# Autodesk Inventor assembly: 00_X02598_LEGOmini_CityGuy
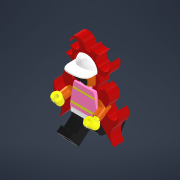
[picture p0: Inventor's stored thumbnail of the model, 180x180]
Saved by Autodesk Inventor 2022 (Build 260153000, 153)
## iProperties
Created: 2022-02-05
Part Number: 00_X02598_LEGOmini_CityGuy
Document SubType Name: Assembly
Designer: Jason
Author: Jason
## Documents named in this file (5)
- C:\Users\User\Desktop\教材_LEGOmini_2022_20220218\00_X02598_LEGOmini_CityGuy.iam
- C:\Users\User\Desktop\教材_LEGOmini_2022_20220218\X02598_LEGOmini_LowerBody.iam
- C:\Users\User\Desktop\教材_LEGOmini_2022_20220218\X02598_LEGOmini_UpperBody.iam
- C:\Users\User\Desktop\教材_LEGOmini_2022_20220218\X02598_LEGOmini_Head_Y.ipt
- C:\Users\User\Desktop\教材_LEGOmini_2022_20220218\X02598_LEGOmini_Hat_R.ipt
## Components (4 placed, 4 different names)
1. X02598_LEGOmini_LowerBody:1 [sub-assembly] — 貼合:1, 齊平:1, 齊平:2
2. X02598_LEGOmini_UpperBody:1 [sub-assembly] — 貼合:1, 齊平:1, 齊平:2, 插入:1, 齊平:3
3. X02598_LEGOmini_Head_Y:1 — 插入:1, 插入:2, 齊平:3
4. X02598_LEGOmini_Hat_R:1 — 插入:2
## Relationships (6: Flush 3, Insert 2, Mate 1)
- 貼合:1 [Mate]: X02598_LEGOmini_LowerBody:1 ↔ X02598_LEGOmini_UpperBody:1
- 齊平:1 [Flush]: X02598_LEGOmini_LowerBody:1 ↔ X02598_LEGOmini_UpperBody:1
- 齊平:2 [Flush]: X02598_LEGOmini_LowerBody:1 ↔ X02598_LEGOmini_UpperBody:1
- 插入:1 [Insert]: X02598_LEGOmini_UpperBody:1 ↔ X02598_LEGOmini_Head_Y:1
- 插入:2 [Insert]: X02598_LEGOmini_Head_Y:1 ↔ X02598_LEGOmini_Hat_R:1
- 齊平:3 [Flush]: X02598_LEGOmini_UpperBody:1 ↔ X02598_LEGOmini_Head_Y:1
